# Autodesk Inventor assembly: Mini Wheel and Bearings
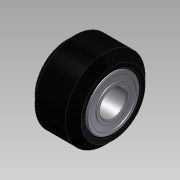
[picture p0: Inventor's stored thumbnail of the model, 180x180]
Saved by Autodesk Inventor 2013 SP2 (Build 170200200, 200)
## iProperties
Created: 2013-06-21
Part Number: Mini Wheel and Bearings
Document SubType Name: Assembly
Designer: Jon Hollander
Author: Jon Hollander
## Documents named in this file (4)
- F:\Dropbox\Research\Loom\Loom Vault\Libary Import\Mini V Carriage\Mini Wheel and Bearings.iam
- C:\Users\Jon Hollander\Documents\Inventor\Content Center Files\R2013\en-US\Micro V Wheel\Micro V Wheel.ipt
- F:\Dropbox\Research\Loom\Loom Vault\Libary Import\Mini V Carriage\WML5010ZZ.iam
- C:\Users\Jon Hollander\Documents\Inventor\Content Center Files\R2013\en-US\Micro V Precision Shim\Micro V Precision Shim.ipt
## Components (4 placed, 3 different names)
1. Micro V Wheel Micro V Wheel:1 — Mate:1, Mate:2, Mate:4
2. WML5010ZZ:1 [sub-assembly] — Mate:1, Mate:2, Mate:5, Mate:6
3. WML5010ZZ:2 [sub-assembly] — Mate:4, Mate:7
4. Micro V Precision Shim Micro V Precision Shim:1 — Mate:5, Mate:6, Mate:7
## Relationships (6: Mate 6)
- Mate:1: Micro V Wheel Micro V Wheel:1 ↔ WML5010ZZ:1
- Mate:2: Micro V Wheel Micro V Wheel:1 ↔ WML5010ZZ:1
- Mate:4: Micro V Wheel Micro V Wheel:1 ↔ WML5010ZZ:2
- Mate:5: WML5010ZZ:1 ↔ Micro V Precision Shim Micro V Precision Shim:1
- Mate:6: WML5010ZZ:1 ↔ Micro V Precision Shim Micro V Precision Shim:1
- Mate:7: WML5010ZZ:2 ↔ Micro V Precision Shim Micro V Precision Shim:1
